# Autodesk Inventor assembly: Collector Arms v2.0_MIR
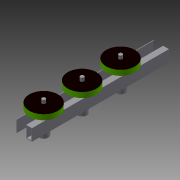
[picture p0: Inventor's stored thumbnail of the model, 180x180]
Saved by Autodesk Inventor 2015 (Build 190159000, 159)
## iProperties
Created: 2015-01-20
Part Number: Collector Arms v2.0_MIR
Document SubType Name: Assembly
Designer: chapale16
Author: chapale16
## Documents named in this file (5)
- \\lhssvr02\Homedirs\Robotics Club\CAD Model 2015\Game Components\The Tote Collector-Arms\Collector Arms v2.0_MIR.iam
- \\lhssvr02\Homedirs\Robotics Club\CAD Model 2015\Game Components\The Tote Collector-Arms\23.5 in 2 x 1 boxBeam_MIR.ipt
- \\lhssvr02\Homedirs\Robotics Club\CAD Model 2015\Game Components\The Tote Collector-Arms\23.5 sheet metal_MIR.ipt
- \\lhssvr02\Homedirs\Robotics Club\CAD Model 2015\Game Components\The Tote Collector-Arms\P60 Gear Box_MIR2.ipt
- \\lhssvr02\Homedirs\Robotics Club\CAD Model 2015\Game Components\The Tote Collector-Arms\collector arm wheel_MIR2.ipt
## Components (8 placed, 4 different names)
1. 23.5 in 2 x 1 boxBeam_MIR:1 — Flush:8, Flush:7, Flush:2, Mate:1, Flush:1, Flush:3, Mate:5, Flush:5, Mate:8
2. 23.5 sheet metal_MIR:1 — Flush:8, Flush:7, Mate:9
3. P60 Gear Box_MIR2:1 — Mate:9, Flush:2, Mate:1, Flush:1, Mate:2, Mate:4
4. collector arm wheel_MIR2:1 — Mate:2, Flush:4
5. P60 Gear Box_MIR2:2 — Flush:3, Mate:5, Mate:4, Mate:3, Mate:7
6. collector arm wheel_MIR2:2 — Flush:4, Mate:3, Flush:6
7. P60 Gear Box_MIR2:3 — Flush:5, Mate:8, Mate:7, Mate:6
8. collector arm wheel_MIR2:3 — Flush:6, Mate:6
## Relationships (17: Mate 9, Flush 8)
- Flush:8: 23.5 in 2 x 1 boxBeam_MIR:1 ↔ 23.5 sheet metal_MIR:1
- Flush:7: 23.5 in 2 x 1 boxBeam_MIR:1 ↔ 23.5 sheet metal_MIR:1
- Mate:9: 23.5 sheet metal_MIR:1 ↔ P60 Gear Box_MIR2:1
- Flush:2 (144.8308 mm): 23.5 in 2 x 1 boxBeam_MIR:1 ↔ P60 Gear Box_MIR2:1
- Mate:1: 23.5 in 2 x 1 boxBeam_MIR:1 ↔ P60 Gear Box_MIR2:1
- Flush:1: 23.5 in 2 x 1 boxBeam_MIR:1 ↔ P60 Gear Box_MIR2:1
- Mate:2: P60 Gear Box_MIR2:1 ↔ collector arm wheel_MIR2:1
- Flush:3: 23.5 in 2 x 1 boxBeam_MIR:1 ↔ P60 Gear Box_MIR2:2
- Mate:5: 23.5 in 2 x 1 boxBeam_MIR:1 ↔ P60 Gear Box_MIR2:2
- Mate:4 (127 mm): P60 Gear Box_MIR2:1 ↔ P60 Gear Box_MIR2:2
- Flush:4: collector arm wheel_MIR2:1 ↔ collector arm wheel_MIR2:2
- Mate:3: P60 Gear Box_MIR2:2 ↔ collector arm wheel_MIR2:2
- Flush:5: 23.5 in 2 x 1 boxBeam_MIR:1 ↔ P60 Gear Box_MIR2:3
- Mate:8: 23.5 in 2 x 1 boxBeam_MIR:1 ↔ P60 Gear Box_MIR2:3
- Mate:7 (127 mm): P60 Gear Box_MIR2:2 ↔ P60 Gear Box_MIR2:3
- Flush:6: collector arm wheel_MIR2:2 ↔ collector arm wheel_MIR2:3
- Mate:6: P60 Gear Box_MIR2:3 ↔ collector arm wheel_MIR2:3
